# Autodesk Inventor assembly: palec
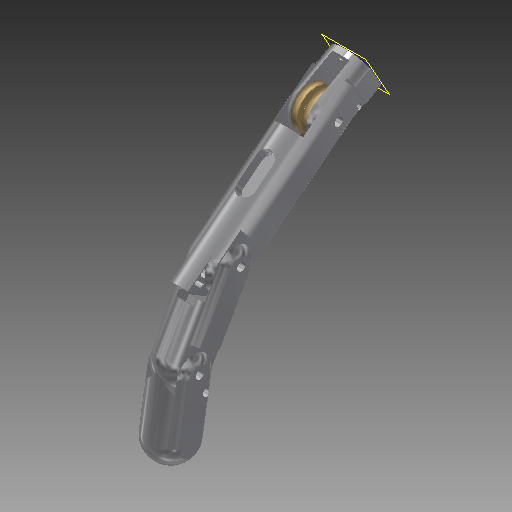
[picture p0: Inventor's stored thumbnail of the model, 512x512]
Saved by Autodesk Inventor 2019 (Build 230136000, 136)
## iProperties
Created: 2019-11-26
Part Number: palec
Document SubType Name: Assembly
Designer: Administrator
Title: Finger all pieces assembled v10
Author: Administrator
## Documents named in this file (7)
- C:\Users\Karolina\Desktop\Kuba\rekav2\palec\palec.iam
- C:\Users\Karolina\Desktop\Kuba\rekav2\palec\Base.ipt
- C:\Users\Karolina\Desktop\Kuba\rekav2\palec\Body.ipt
- C:\Users\Karolina\Desktop\Kuba\rekav2\palec\Middle.ipt
- C:\Users\Karolina\Desktop\Kuba\rekav2\palec\Tip.ipt
- C:\Users\Karolina\Desktop\Kuba\rekav2\palec\Lever korekta.ipt
- C:\Users\Karolina\Desktop\Kuba\rekav2\palec\Pullie.ipt
## Components (7 placed, 6 different names)
1. Base:1 — Zestawiający:1, Zestawiający:2, Zestawiający:9, Zestawiający:10, Zestawiający:11
2. Body:1 — Zestawiający:1, Zestawiający:2, Zestawiający:14, Zestawiający:15, Zestawiający:16, Zestawiający:17
3. Middle:1 — Zestawiający:7, Zestawiający:8, Zestawiający:9, Zestawiający:10, Zestawiający:13
4. Tip:1 — Zestawiający:7, Zestawiający:8, Zestawiający:12
5. Lever korekta:1 — Zestawiający:11, Zestawiający:12, Zestawiający:13
6. Pullie:1 — Zestawiający:14, Zestawiający:15
7. Pullie:2 — Zestawiający:16, Zestawiający:17
## Relationships (13: Mate 13)
- Zestawiający:1 [Mate]: Base:1 ↔ Body:1
- Zestawiający:2 [Mate]: Base:1 ↔ Body:1
- Zestawiający:7 [Mate]: Middle:1 ↔ Tip:1
- Zestawiający:8 [Mate]: Middle:1 ↔ Tip:1
- Zestawiający:9 [Mate]: Base:1 ↔ Middle:1
- Zestawiający:10 [Mate]: Base:1 ↔ Middle:1
- Zestawiający:11 [Mate]: Base:1 ↔ Lever korekta:1
- Zestawiający:12 [Mate]: Tip:1 ↔ Lever korekta:1
- Zestawiający:13 [Mate]: Middle:1 ↔ Lever korekta:1
- Zestawiający:14 [Mate]: Body:1 ↔ Pullie:1
- Zestawiający:15 [Mate]: Body:1 ↔ Pullie:1
- Zestawiający:16 [Mate]: Body:1 ↔ Pullie:2
- Zestawiający:17 [Mate]: Body:1 ↔ Pullie:2
